# Autodesk Inventor assembly: Vise_final
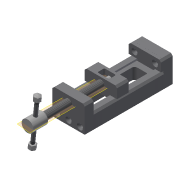
[picture p0: Inventor's stored thumbnail of the model, 180x180]
Saved by Autodesk Inventor 2022 Beta2 (Build 260130000, 130) ContinuousBuild 0
## iProperties
Created: 2011-03-10
Part Number: Vise_final
Document SubType Name: Assembly
Designer: jmacmillan
Author: jmacmillan
## Documents named in this file (7)
- C:\Autodesk Inventor 2021 Intro Practice Files\Vise_final.iam
- C:\Autodesk Inventor 2021 Intro Practice Files\Body.ipt
- C:\Autodesk Inventor 2021 Intro Practice Files\MovingJaw.ipt
- C:\Autodesk Inventor 2021 Intro Practice Files\Spindle.ipt
- C:\Autodesk Inventor 2021 Intro Practice Files\Pin.ipt
- C:\Autodesk Inventor 2021 Intro Practice Files\FixedJaw.ipt
- C:\Autodesk Inventor 2021 Intro Practice Files\DIN 917 - M6 x 1 10 copy.ipt
## Components (7 placed, 6 different names)
1. Body:1 — Mate:1, Mate:6, Flush:2, Insert:3, Flush:3
2. MovingJaw:1 — Mate:1, Mate:6, Flush:2, Insert:4
3. Spindle:1 — Insert:4, Mate:2, Mate:3
4. Pin:1 — Mate:2, Mate:3, Mate:4, Mate:5, Insert:2
5. DIN 917 M6:3 — Mate:4, Mate:5
6. DIN 917 M6:4 — Insert:2
7. FixedJaw:1 — Insert:3, Flush:3
## Relationships (11: Mate 6, Insert 3, Flush 2)
- Mate:1: Body:1 ↔ MovingJaw:1
- Mate:6 (40 mm): Body:1 ↔ MovingJaw:1
- Flush:2: Body:1 ↔ MovingJaw:1
- Insert:4: MovingJaw:1 ↔ Spindle:1
- Mate:2: Spindle:1 ↔ Pin:1
- Mate:3: Spindle:1 ↔ Pin:1
- Mate:5 (-6.5 mm): Pin:1 ↔ DIN 917 M6:3
- Insert:2 (-6.5 mm): Pin:1 ↔ DIN 917 M6:4
- Insert:3: Body:1 ↔ FixedJaw:1
- Flush:3: Body:1 ↔ FixedJaw:1
- Mate:4: Pin:1 ↔ DIN 917 M6:3
